# Autodesk Inventor assembly: J0_Drive
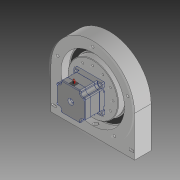
[picture p0: Inventor's stored thumbnail of the model, 180x180]
Saved by Autodesk Inventor 2020 (Build 240168000, 168)
## iProperties
Created: 2021-03-20
Part Number: J0_Drive
Document SubType Name: Assembly
Designer: DDeGo
Author: DDeGo
## Documents named in this file (6)
- C:\Users\DDeGo\Documents\Drew\Projects\OS-ARM\cad\FirstDraft\J0_Drive.iam
- C:\Users\DDeGo\Documents\Drew\Projects\OS-ARM\cad\OTS\6820 bearing.ipt
- C:\Users\DDeGo\Documents\Drew\Projects\OS-ARM\cad\HarmonicDrive\HarmonicDrive.iam
- C:\Users\DDeGo\Documents\Drew\Projects\OS-ARM\cad\FirstDraft\J0_drivebracket.ipt
- C:\Users\DDeGo\Documents\Drew\Projects\OS-ARM\cad\FirstDraft\J0_motorbracket.ipt
- C:\Users\DDeGo\Documents\Drew\Projects\OS-ARM\cad\OTS\NEMA 23 - 41mm.ipt
## Components (5 placed, 5 different names)
1. 6820 bearing:1 — Mate:1, Mate:2, Mate:3, Mate:12
2. HarmonicDrive:1 [sub-assembly] — Mate:3, Mate:7, Mate:12
3. J0_drivebracket:1 — Mate:1, Angle:1, Mate:2, Mate:5, Mate:6, Mate:8
4. J0_motorbracket:1 — Mate:5, Mate:6, Mate:7, Mate:8, Mate:9, Mate:10, Mate:11
5. NEMA 23 - 41mm:1 — Mate:9, Mate:10, Mate:11
## Relationships (12: Mate 11, Angle 1)
- Mate:1: 6820 bearing:1 ↔ J0_drivebracket:1
- Angle:1 (180 deg): J0_drivebracket:1
- Mate:2: 6820 bearing:1 ↔ J0_drivebracket:1
- Mate:3: 6820 bearing:1 ↔ HarmonicDrive:1
- Mate:5: J0_drivebracket:1 ↔ J0_motorbracket:1
- Mate:6: J0_drivebracket:1 ↔ J0_motorbracket:1
- Mate:7: HarmonicDrive:1 ↔ J0_motorbracket:1
- Mate:8: J0_drivebracket:1 ↔ J0_motorbracket:1
- Mate:9: J0_motorbracket:1 ↔ NEMA 23 - 41mm:1
- Mate:10: J0_motorbracket:1 ↔ NEMA 23 - 41mm:1
- Mate:11: J0_motorbracket:1 ↔ NEMA 23 - 41mm:1
- Mate:12: 6820 bearing:1 ↔ HarmonicDrive:1
